# Autodesk Inventor assembly: middle gear
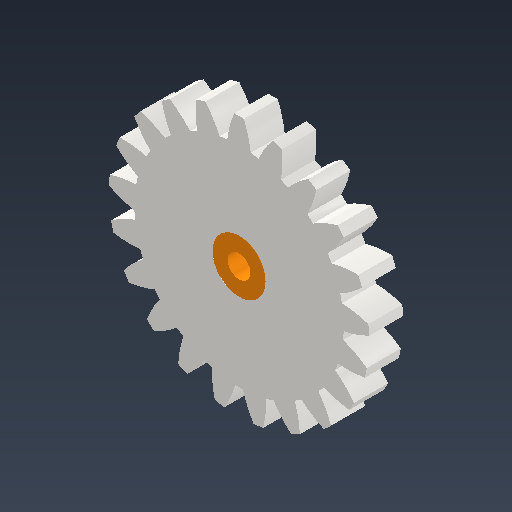
[picture p0: Inventor's stored thumbnail of the model, 512x512]
Saved by Autodesk Inventor 2025.3 (Build 293356000, 356)
## iProperties
Created: 2025-10-14
Part Number: middle gear
Document SubType Name: Assembly
Designer: 陳泓任
Author: 陳泓任
## Documents named in this file (3)
- C:\Users\Ou918\3D-model-temp\introduction to mechanical engineering(1)\middle gear.iam
- C:\Users\Ou918\3D-model-temp\introduction to mechanical engineering(1)\sleeve.ipt
- C:\Users\Ou918\3D-model-temp\introduction to mechanical engineering(1)\version_5\big_gear_pair\機械便覽魔法師\正齒輪21.ipt
## Components (2 placed, 2 different names)
1. sleeve:1 — 貼合:1, 齊平:1
2. 正齒輪2:1 — 貼合:1, 齊平:1
## Relationships (2: Mate 1, Flush 1)
- 貼合:1 [Mate]: sleeve:1 ↔ 正齒輪2:1
- 齊平:1 [Flush]: sleeve:1 ↔ 正齒輪2:1
